# Autodesk Inventor assembly: Assembly_Cube_Lens_holder_CylindricalLens
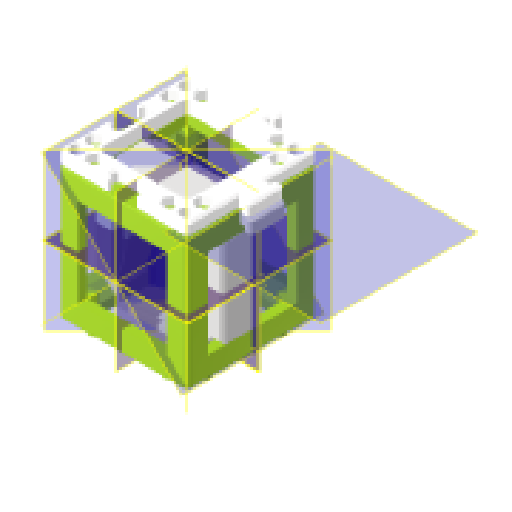
[picture p0: Inventor's stored thumbnail of the model, 512x512]
Saved by Autodesk Inventor 2025.1 (Build 291241020, 241B)
## iProperties
Created: 2020-11-11
Part Number: Assembly_Cube_Lens_holder_CylindricalLens
Document SubType Name: Assembly
Designer: marsikovabarbora
Author: marsikovabarbora
## Documents named in this file (3)
- C:\Users\diederichbenedict\Dropbox\Dokumente\Promotion\PROJECTS\openUC2-CAD\INVENTOR\Assembly_Cube_Lens_holder_CylindricalLens.iam
- C:\Users\diederichbenedict\Dropbox\Dokumente\Promotion\PROJECTS\openUC2-CAD\INVENTOR\Assembly_Cube_empty_IM_v3.iam
- C:\Users\diederichbenedict\Dropbox\Dokumente\Promotion\PROJECTS\openUC2-CAD\INVENTOR\20_Cube_Insert_Lens_Cylindrical_Comar_v3.ipt
## Components (2 placed, 2 different names)
1. Assembly_Cube_empty_IM_v3:1 [sub-assembly] — Mate:1, Mate:2, Mate:3, Flush:1, Flush:2
2. 20_Cube_Insert_Lens_Cylindrical_Comar_v3:1 — Flush:1, Flush:2
## Relationships (5: Mate 3, Flush 2)
- Mate:1: Assembly_Cube_empty_IM_v3:1
- Mate:2: Assembly_Cube_empty_IM_v3:1
- Mate:3: Assembly_Cube_empty_IM_v3:1
- Flush:1: Assembly_Cube_empty_IM_v3:1 ↔ 20_Cube_Insert_Lens_Cylindrical_Comar_v3:1
- Flush:2: Assembly_Cube_empty_IM_v3:1 ↔ 20_Cube_Insert_Lens_Cylindrical_Comar_v3:1
